# Autodesk Inventor assembly: assembly
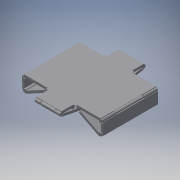
[picture p0: Inventor's stored thumbnail of the model, 180x180]
Saved by Autodesk Inventor 2019 (Build 230136000, 136)
## iProperties
Created: 2018-07-23
Part Number: assembly
Document SubType Name: Assembly
Designer: Ge Shi
Author: Ge Shi
## Documents named in this file (8)
- D:\hive\projects\foldingBaby\v2\assembly.iam
- D:\hive\projects\foldingBaby\v2\backPlate.ipt
- D:\hive\projects\foldingBaby\v2\prototype2dims.ipt
- D:\hive\projects\foldingBaby\v2\topBottomPlate.ipt
- D:\hive\projects\foldingBaby\v2\leftRightPlate.ipt
- D:\hive\projects\foldingBaby\v2\outerFrontPlate.ipt
- D:\hive\projects\foldingBaby\v2\innerFrontPlate.ipt
- D:\hive\projects\foldingBaby\v2\innerLeftRightPlate.ipt
## Components (12 placed, 7 different names)
1. backPlate:1 — Flush:1, Mate:4, Mate:7, Flush:8, Flush:9, Flush:10, Flush:11, Mate:20, Mate:22
2. prototype2dims:1 — Mate:1, Mate:2, Flush:1, Mate:4, Flush:2, Flush:3, Mate:7, Mate:9, Mate:10, Mate:13, Flush:4, Flush:5, Flush:6, Mate:19, Flush:7
3. topBottomPlate:1 — Flush:2, Flush:10, Mate:22, Mate:23
4. topBottomPlate:2 — Flush:3, Flush:11, Mate:20, Mate:21
5. leftRightPlate:1 — Mate:9, Flush:8
6. leftRightPlate:2 — Mate:10, Flush:9
7. outerFrontPlate:1 — Mate:13, Mate:23
8. outerFrontPlate:2 — Flush:4, Mate:21
9. innerFrontPlate:1 — Flush:5
10. innerFrontPlate:2 — Flush:6
11. innerLeftRightPlate:1 — Mate:19
12. innerLeftRightPlate:2 — Flush:7
## Relationships (23: Mate 12, Flush 11)
- Mate:1: prototype2dims:1
- Mate:2: prototype2dims:1
- Flush:1: backPlate:1 ↔ prototype2dims:1
- Mate:4 (50 mm): backPlate:1 ↔ prototype2dims:1
- Flush:2: prototype2dims:1 ↔ topBottomPlate:1
- Flush:3: prototype2dims:1 ↔ topBottomPlate:2
- Mate:7: backPlate:1 ↔ prototype2dims:1
- Mate:9: prototype2dims:1 ↔ leftRightPlate:1
- Mate:10: prototype2dims:1 ↔ leftRightPlate:2
- Mate:13: prototype2dims:1 ↔ outerFrontPlate:1
- Flush:4: prototype2dims:1 ↔ outerFrontPlate:2
- Flush:5: prototype2dims:1 ↔ innerFrontPlate:1
- Flush:6: prototype2dims:1 ↔ innerFrontPlate:2
- Mate:19: prototype2dims:1 ↔ innerLeftRightPlate:1
- Flush:7: prototype2dims:1 ↔ innerLeftRightPlate:2
- Flush:8: backPlate:1 ↔ leftRightPlate:1
- Flush:9: backPlate:1 ↔ leftRightPlate:2
- Flush:10: backPlate:1 ↔ topBottomPlate:1
- Flush:11: backPlate:1 ↔ topBottomPlate:2
- Mate:20: backPlate:1 ↔ topBottomPlate:2
- Mate:21: topBottomPlate:2 ↔ outerFrontPlate:2
- Mate:22: backPlate:1 ↔ topBottomPlate:1
- Mate:23: topBottomPlate:1 ↔ outerFrontPlate:1
## Named parameters: length = 50 mm, width = 40 mm, height = 100 mm, hingeShaft = 3 mm, clearance = 1.5 mm, thick = 4 mm, hingeShaftMidLen = 0.5, hingeShaftHolder = 5.5 mm
